# Autodesk Inventor assembly: Boot
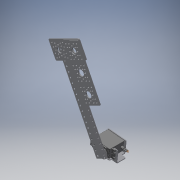
[picture p0: Inventor's stored thumbnail of the model, 180x180]
Saved by Autodesk Inventor 2017 (Build 210142000, 142)
## iProperties
Created: 2017-03-23
Part Number: Boot
Document SubType Name: Assembly
Designer: User
Author: User
## Documents named in this file (6)
- C:\Robotics\CAD\2016-17_CAD\Boot.iam
- C:\Robotics\CAD\COTSParts\Tetrix\Tetrix bracket - single servo.ipt
- C:\Robotics\CAD\COTSParts\Tetrix\Tetrix servo 180.ipt
- C:\Robotics\CAD\COTSParts\Actobotics\585 parts\585396.ipt
- C:\Robotics\CAD\COTSParts\Actobotics\585 parts\585422.ipt
- C:\Robotics\CAD\COTSParts\Actobotics\585 parts\585580.ipt
## Components (5 placed, 5 different names)
1. Tetrix bracket - single servo:1 — Flush:1, Flush:2, Mate:1, Flush:3
2. Tetrix servo 180:1 — Flush:1, Flush:2, Mate:1, Flush:3, Insert:1
3. 585396:1 — Insert:1, Insert:2, Flush:4
4. 585422:1 — Insert:2, Flush:4, Insert:3, Insert:4
5. 585580:1 — Insert:3, Insert:4
## Relationships (9: Flush 4, Insert 4, Mate 1)
- Flush:1 (0.508 mm): Tetrix bracket - single servo:1 ↔ Tetrix servo 180:1
- Flush:2 (0.508 mm): Tetrix bracket - single servo:1 ↔ Tetrix servo 180:1
- Mate:1: Tetrix bracket - single servo:1 ↔ Tetrix servo 180:1
- Flush:3 (3.5052 mm): Tetrix bracket - single servo:1 ↔ Tetrix servo 180:1
- Insert:1: Tetrix servo 180:1 ↔ 585396:1
- Insert:2: 585396:1 ↔ 585422:1
- Flush:4 (4.7244 mm): 585396:1 ↔ 585422:1
- Insert:3: 585422:1 ↔ 585580:1
- Insert:4: 585422:1 ↔ 585580:1
